# Autodesk Inventor assembly: Lensfree_flexstage_box
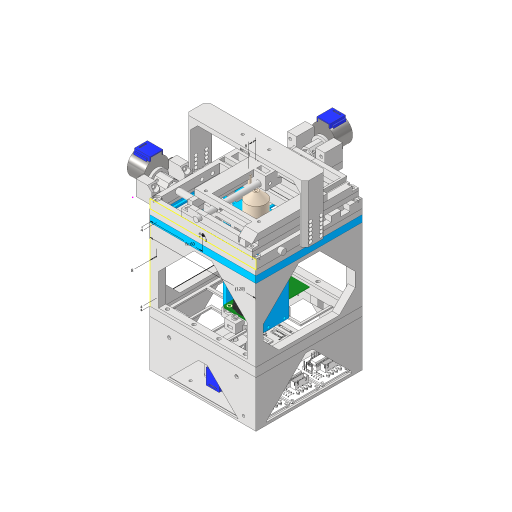
[picture p0: Inventor's stored thumbnail of the model, 512x512]
Saved by Autodesk Inventor 2023 (Build 270158000, 158)
## iProperties
Created: 2020-12-08
Part Number: Lensfree_flexstage_box
Document SubType Name: Assembly
Designer: CDT
Author: CDT
## Documents named in this file (22)
- C:\Users\CDT\OneDrive - University of Glasgow\CDT\Year 2\8. Smartphone conventional microscope\1. Models\41. Smartphone_inverted_small_v8\Lensfree_flexstage_box.iam
- C:\Users\CDT\OneDrive - University of Glasgow\CDT\Year 2\8. Smartphone conventional microscope\1. Models\41. Smartphone_inverted_small_v8\28BYJ-48 Stepper.ipt
- C:\Users\CDT\OneDrive - University of Glasgow\CDT\Year 2\8. Smartphone conventional microscope\1. Models\41. Smartphone_inverted_small_v8\Bottom_carriage.ipt
- C:\Users\CDT\OneDrive - University of Glasgow\CDT\Year 2\8. Smartphone conventional microscope\1. Models\41. Smartphone_inverted_small_v8\ULN2003 Stepper Driver.ipt
- C:\Users\CDT\OneDrive - University of Glasgow\CDT\Year 2\8. Smartphone conventional microscope\1. Models\41. Smartphone_inverted_small_v8\160mm_shunt_box.ipt
- C:\Users\CDT\OneDrive - University of Glasgow\CDT\Year 2\8. Smartphone conventional microscope\1. Models\41. Smartphone_inverted_small_v8\Raspberry Pi HQ Camera.ipt
- C:\Users\CDT\OneDrive - University of Glasgow\CDT\Year 2\8. Smartphone conventional microscope\1. Models\41. Smartphone_inverted_small_v8\AC127-075-A-Step.ipt
- C:\Users\CDT\OneDrive - University of Glasgow\CDT\Year 2\8. Smartphone conventional microscope\1. Models\41. Smartphone_inverted_small_v8\Flexible_tube_bolster_fixed_v3.ipt
- C:\Users\CDT\OneDrive - University of Glasgow\CDT\Year 2\8. Smartphone conventional microscope\1. Models\41. Smartphone_inverted_small_v8\Objective_placeholder_V2.ipt
- C:\Users\CDT\OneDrive - University of Glasgow\CDT\Year 2\8. Smartphone conventional microscope\1. Models\41. Smartphone_inverted_small_v8\slide_clips_4mm.ipt
- C:\Users\CDT\OneDrive - University of Glasgow\CDT\Year 2\8. Smartphone conventional microscope\1. Models\41. Smartphone_inverted_small_v8\Flexible_cam_holder_v7_HQ.ipt
- C:\Users\CDT\OneDrive - University of Glasgow\CDT\Year 2\8. Smartphone conventional microscope\1. Models\41. Smartphone_inverted_small_v8\RapberryPiZero.ipt
- C:\Users\CDT\OneDrive - University of Glasgow\CDT\Year 2\8. Smartphone conventional microscope\1. Models\41. Smartphone_inverted_small_v8\Tube_lens_holder.ipt
- C:\Users\CDT\OneDrive - University of Glasgow\CDT\Year 2\8. Smartphone conventional microscope\1. Models\41. Smartphone_inverted_small_v8\3mm_shaft_couple_sideclip_v4.ipt
- C:\Users\CDT\OneDrive - University of Glasgow\CDT\Year 2\8. Smartphone conventional microscope\1. Models\41. Smartphone_inverted_small_v8\6mm_shaft_couple_sideclip_v2.ipt
- C:\Users\CDT\OneDrive - University of Glasgow\CDT\Year 2\8. Smartphone conventional microscope\1. Models\41. Smartphone_inverted_small_v8\Rail_stage_x_m6_v2.ipt
- C:\Users\CDT\OneDrive - University of Glasgow\CDT\Year 2\8. Smartphone conventional microscope\1. Models\41. Smartphone_inverted_small_v8\Rail_carriage_v2.ipt
- C:\Users\CDT\OneDrive - University of Glasgow\CDT\Year 2\8. Smartphone conventional microscope\1. Models\41. Smartphone_inverted_small_v8\Rail_stage_y_v1.ipt
- C:\Users\CDT\OneDrive - University of Glasgow\CDT\Year 2\8. Smartphone conventional microscope\1. Models\41. Smartphone_inverted_small_v8\Led_frame_2_4mm.ipt
- C:\Users\CDT\OneDrive - University of Glasgow\CDT\Year 2\8. Smartphone conventional microscope\1. Models\41. Smartphone_inverted_small_v8\Rail_carriage_y_top_v2.ipt
- C:\Users\CDT\OneDrive - University of Glasgow\CDT\Year 2\8. Smartphone conventional microscope\1. Models\41. Smartphone_inverted_small_v8\Stage_shunt.ipt
- C:\Users\CDT\OneDrive - University of Glasgow\CDT\Year 2\6. LED Matrix lensfree\1. Models\45. Arducam_Lensfree_Fibrehead_V21\M6 Screw.ipt
## Components (27 placed, 21 different names)
1. 28BYJ-48 Stepper:7 — Mate:430, Mate:431, Mate:432, Mate:437
2. 28BYJ-48 Stepper:8 — Mate:427, Mate:428, Mate:429, Mate:436
3. Tube_lens_holder:1 — Mate:283, Mate:295, Mate:307
4. Objective_placeholder_V2:1 — Mate:238, Mate:287
5. Flexible_tube_bolster_fixed_v3:1 — Mate:238, Mate:239, Mate:283, Mate:287, Flush:92, Mate:288, Mate:295, Flush:127, Flush:128, Flush:129
6. Raspberry Pi HQ Camera:2 — Mate:420, Mate:421, Mate:422
7. AC127-075-A-Step:1 — Mate:239, Mate:307
8. 160mm_shunt_box:1 — Flush:92, Mate:288, Flush:127, Mate:423, Mate:424, Flush:130, Mate:426
9. 28BYJ-48 Stepper:9 — Mate:297, Mate:298, Mate:299, Mate:349, Mate:350, Mate:351, Mate:352
10. RapberryPiZero:1 — Mate:303, Mate:304, Mate:305
11. ULN2003 Stepper Driver:2 — Mate:61, Mate:62, Mate:63
12. ULN2003 Stepper Driver:3 — Mate:66, Mate:117
13. ULN2003 Stepper Driver:1 — Mate:58, Mate:72, Mate:73
14. M6 Screw:1 — Mate:439, Mate:440
15. M6 Screw:2 — Mate:441, Mate:442
16. 6mm_shaft_couple_sideclip_v2:2 — Mate:437, Mate:438, Mate:442
17. Stage_shunt:1 — Flush:128, Flush:129, Flush:130, Mate:425, Flush:131, Flush:132
18. Rail_carriage_y_top_v2:1 — Flush:124, Mate:419
19. Rail_carriage_v2:1 — Mate:412, Flush:118, Flush:120, Mate:414, Flush:121
20. Rail_stage_x_m6_v2:1 — Mate:412, Flush:118, Mate:425, Flush:131, Flush:132, Mate:427, Mate:428, Mate:429, Mate:433, Mate:434, Mate:435, Mate:440
21. Rail_stage_y_v1:1 — Flush:120, Mate:414, Flush:121, Flush:124, Mate:419, Mate:430, Mate:431, Mate:432, Mate:438, Mate:441
22. Led_frame_2_4mm:1 — Mate:433, Mate:434
23. 6mm_shaft_couple_sideclip_v2:1 — Mate:435, Mate:436, Mate:439
24. 3mm_shaft_couple_sideclip_v4:2 — Mate:349, Mate:350, Mate:352
25. Flexible_cam_holder_v7_HQ:2 — Flush:108, Flush:109, Mate:364, Mate:420, Mate:421, Mate:422, Mate:423, Mate:424, Mate:426
26. slide_clips_4mm:1
27. Bottom_carriage:1 — Mate:58, Mate:61, Mate:62, Mate:63, Mate:66, Mate:72, Mate:73, Mate:117, Mate:297, Mate:298, Mate:299, Mate:303, Mate:304, Mate:305, Mate:351, Flush:108, Flush:109, Mate:364
## Relationships (65: Mate 52, Flush 13)
- Mate:58 (1 mm): ULN2003 Stepper Driver:1 ↔ Bottom_carriage:1
- Mate:61: ULN2003 Stepper Driver:2 ↔ Bottom_carriage:1
- Mate:62: ULN2003 Stepper Driver:2 ↔ Bottom_carriage:1
- Mate:63: ULN2003 Stepper Driver:2 ↔ Bottom_carriage:1
- Mate:66: ULN2003 Stepper Driver:3 ↔ Bottom_carriage:1
- Mate:72: ULN2003 Stepper Driver:1 ↔ Bottom_carriage:1
- Mate:73: ULN2003 Stepper Driver:1 ↔ Bottom_carriage:1
- Mate:117: ULN2003 Stepper Driver:3 ↔ Bottom_carriage:1
- Mate:238: Objective_placeholder_V2:1 ↔ Flexible_tube_bolster_fixed_v3:1
- Mate:239: Flexible_tube_bolster_fixed_v3:1 ↔ AC127-075-A-Step:1
- Mate:283: Tube_lens_holder:1 ↔ Flexible_tube_bolster_fixed_v3:1
- Mate:287 (-2.25 mm): Objective_placeholder_V2:1 ↔ Flexible_tube_bolster_fixed_v3:1
- Flush:92: Flexible_tube_bolster_fixed_v3:1 ↔ 160mm_shunt_box:1
- Mate:288: Flexible_tube_bolster_fixed_v3:1 ↔ 160mm_shunt_box:1
- Mate:295: Tube_lens_holder:1 ↔ Flexible_tube_bolster_fixed_v3:1
- Mate:297: 28BYJ-48 Stepper:9 ↔ Bottom_carriage:1
- Mate:298: 28BYJ-48 Stepper:9 ↔ Bottom_carriage:1
- Mate:299: 28BYJ-48 Stepper:9 ↔ Bottom_carriage:1
- Mate:303: RapberryPiZero:1 ↔ Bottom_carriage:1
- Mate:304: RapberryPiZero:1 ↔ Bottom_carriage:1
- Mate:305: RapberryPiZero:1 ↔ Bottom_carriage:1
- Mate:307 (-135 mm): Tube_lens_holder:1 ↔ AC127-075-A-Step:1
- Mate:349: 28BYJ-48 Stepper:9 ↔ 3mm_shaft_couple_sideclip_v4:2
- Mate:350: 28BYJ-48 Stepper:9 ↔ 3mm_shaft_couple_sideclip_v4:2
- Mate:351: 28BYJ-48 Stepper:9 ↔ Bottom_carriage:1
- Mate:352: 28BYJ-48 Stepper:9 ↔ 3mm_shaft_couple_sideclip_v4:2
- Flush:108: Flexible_cam_holder_v7_HQ:2 ↔ Bottom_carriage:1
- Flush:109: Flexible_cam_holder_v7_HQ:2 ↔ Bottom_carriage:1
- Mate:364: Flexible_cam_holder_v7_HQ:2 ↔ Bottom_carriage:1
- Mate:412 (0.1 mm): Rail_carriage_v2:1 ↔ Rail_stage_x_m6_v2:1
- Flush:118: Rail_carriage_v2:1 ↔ Rail_stage_x_m6_v2:1
- Flush:120: Rail_carriage_v2:1 ↔ Rail_stage_y_v1:1
- Mate:414: Rail_carriage_v2:1 ↔ Rail_stage_y_v1:1
- Flush:121: Rail_carriage_v2:1 ↔ Rail_stage_y_v1:1
- Flush:124: Rail_carriage_y_top_v2:1 ↔ Rail_stage_y_v1:1
- Mate:419: Rail_carriage_y_top_v2:1 ↔ Rail_stage_y_v1:1
- Mate:420: Raspberry Pi HQ Camera:2 ↔ Flexible_cam_holder_v7_HQ:2
- Mate:421: Raspberry Pi HQ Camera:2 ↔ Flexible_cam_holder_v7_HQ:2
- Mate:422: Raspberry Pi HQ Camera:2 ↔ Flexible_cam_holder_v7_HQ:2
- Flush:127: Flexible_tube_bolster_fixed_v3:1 ↔ 160mm_shunt_box:1
- Flush:128: Flexible_tube_bolster_fixed_v3:1 ↔ Stage_shunt:1
- Mate:423: 160mm_shunt_box:1 ↔ Flexible_cam_holder_v7_HQ:2
- Mate:424: 160mm_shunt_box:1 ↔ Flexible_cam_holder_v7_HQ:2
- Flush:129: Flexible_tube_bolster_fixed_v3:1 ↔ Stage_shunt:1
- Flush:130: 160mm_shunt_box:1 ↔ Stage_shunt:1
- Mate:425: Stage_shunt:1 ↔ Rail_stage_x_m6_v2:1
- Flush:131: Stage_shunt:1 ↔ Rail_stage_x_m6_v2:1
- Mate:426: 160mm_shunt_box:1 ↔ Flexible_cam_holder_v7_HQ:2
- Flush:132: Stage_shunt:1 ↔ Rail_stage_x_m6_v2:1
- Mate:427: 28BYJ-48 Stepper:8 ↔ Rail_stage_x_m6_v2:1
- Mate:428: 28BYJ-48 Stepper:8 ↔ Rail_stage_x_m6_v2:1
- Mate:429: 28BYJ-48 Stepper:8 ↔ Rail_stage_x_m6_v2:1
- Mate:430: 28BYJ-48 Stepper:7 ↔ Rail_stage_y_v1:1
- Mate:431: 28BYJ-48 Stepper:7 ↔ Rail_stage_y_v1:1
- Mate:432: 28BYJ-48 Stepper:7 ↔ Rail_stage_y_v1:1
- Mate:433: Rail_stage_x_m6_v2:1 ↔ Led_frame_2_4mm:1
- Mate:434: Rail_stage_x_m6_v2:1 ↔ Led_frame_2_4mm:1
- Mate:435: Rail_stage_x_m6_v2:1 ↔ 6mm_shaft_couple_sideclip_v2:1
- Mate:436: 28BYJ-48 Stepper:8 ↔ 6mm_shaft_couple_sideclip_v2:1
- Mate:437: 28BYJ-48 Stepper:7 ↔ 6mm_shaft_couple_sideclip_v2:2
- Mate:438: 6mm_shaft_couple_sideclip_v2:2 ↔ Rail_stage_y_v1:1
- Mate:439: M6 Screw:1 ↔ 6mm_shaft_couple_sideclip_v2:1
- Mate:440: M6 Screw:1 ↔ Rail_stage_x_m6_v2:1
- Mate:441: M6 Screw:2 ↔ Rail_stage_y_v1:1
- Mate:442: M6 Screw:2 ↔ 6mm_shaft_couple_sideclip_v2:2
